# Autodesk Inventor assembly: Link_01_Assembly_V02
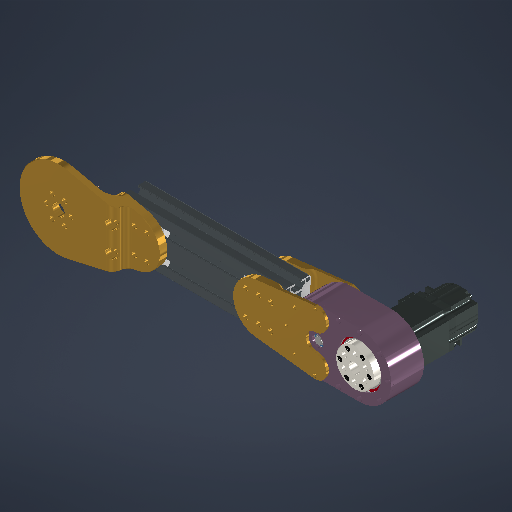
[picture p0: Inventor's stored thumbnail of the model, 512x512]
Saved by Autodesk Inventor 2026 (Build 300175000, 175)
## iProperties
Created: 2025-12-01
Part Number: Link_01_Assembly_V02
Document SubType Name: Assembly
Designer: DanielFGarzon
Mass: 1937.28 g
Surface Area: 3111.54 cm^2
Volume: 616.157 cm^3
Density: 3.14413 g/cm^3
Author: DanielFGarzon
## Documents named in this file (5)
- D:\POLIMI\3RD SEMESTER\Industrial Robotics\Project\Mine\Inventor_Files\Link_01_Assembly_V04.iam
- D:\POLIMI\3RD SEMESTER\Industrial Robotics\Project\Mine\Inventor_Files\RotationalConector_30x60.ipt
- D:\POLIMI\3RD SEMESTER\Industrial Robotics\Project\Mine\Inventor_Files\Link_01_V03.ipt
- D:\POLIMI\3RD SEMESTER\Industrial Robotics\Project\Mine\Inventor_Files\Reducer_02\Reducer_Motor_HG-KR13.iam
- D:\POLIMI\3RD SEMESTER\Industrial Robotics\Project\Mine\Inventor_Files\Reducer_02\RigidConector_30x60_v04.ipt
## Components (5 placed, 4 different names)
1. RotationalConector_30x60:1 — Mate:1, Mate:2, Mate:3, Mate:4
2. Link_01_V03:1 — Mate:2, Mate:3, Mate:4, Flush:2, Mate:15, Mate:16, Mate:17, Mate:18, Mate:19, Mate:20, Mate:21
3. Reducer_Motor_HG-KR13:1 [sub-assembly] — Mate:22, Mate:23, Mate:24
4. RigidConector_30x60_v04:1 — Mate:16, Mate:17, Mate:18, Mate:22, Mate:23, Mate:24
5. RigidConector_30x60_v04:2 — Mate:19, Mate:20, Mate:21
## Relationships (16: Mate 15, Flush 1)
- Mate:1: RotationalConector_30x60:1
- Mate:2: RotationalConector_30x60:1 ↔ Link_01_V03:1
- Mate:3: RotationalConector_30x60:1 ↔ Link_01_V03:1
- Mate:4: RotationalConector_30x60:1 ↔ Link_01_V03:1
- Flush:2 (-30 mm): Link_01_V03:1
- Mate:14
- Mate:15: Link_01_V03:1
- Mate:16: Link_01_V03:1 ↔ RigidConector_30x60_v04:1
- Mate:17: Link_01_V03:1 ↔ RigidConector_30x60_v04:1
- Mate:18: Link_01_V03:1 ↔ RigidConector_30x60_v04:1
- Mate:19: Link_01_V03:1 ↔ RigidConector_30x60_v04:2
- Mate:20: Link_01_V03:1 ↔ RigidConector_30x60_v04:2
- Mate:21: Link_01_V03:1 ↔ RigidConector_30x60_v04:2
- Mate:22: Reducer_Motor_HG-KR13:1 ↔ RigidConector_30x60_v04:1
- Mate:23: Reducer_Motor_HG-KR13:1 ↔ RigidConector_30x60_v04:1
- Mate:24: Reducer_Motor_HG-KR13:1 ↔ RigidConector_30x60_v04:1
